# Autodesk Inventor assembly: ANDGATEASSEMBLY
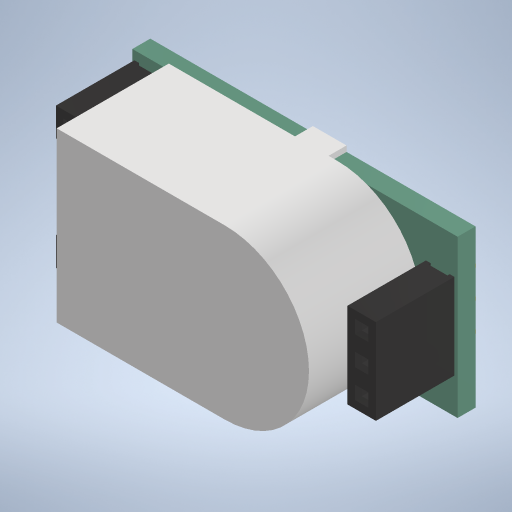
[picture p0: Inventor's stored thumbnail of the model, 512x512]
Saved by Autodesk Inventor 2023 (Build 270158000, 158)
## iProperties
Created: 2024-01-22
Part Number: ANDGATEASSEMBLY
Document SubType Name: Assembly
Designer: Jetsan
Author: Jetsan
## Documents named in this file (3)
- C:\Git\DigitalLogicProject\Gates\ANDGATE\ANDGATEASSEMBLY.iam
- C:\Git\DigitalLogicProject\Gates\ANDGATE\ANDGATE.iam
- C:\Git\DigitalLogicProject\Gates\ANDGATE\ANDGATE.ipt
## Components (2 placed, 1 different names)
1. ANDGATE:1 [sub-assembly] — Mate:1, Mate:4, Mate:5
2. ANDGATE:2 — Mate:1, Mate:4, Mate:5
## Relationships (3: Mate 3)
- Mate:1: ANDGATE:1 ↔ ANDGATE:2
- Mate:4: ANDGATE:1 ↔ ANDGATE:2
- Mate:5: ANDGATE:1 ↔ ANDGATE:2
